# Autodesk Inventor assembly: Asta_verticale
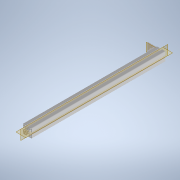
[picture p0: Inventor's stored thumbnail of the model, 180x180]
Saved by Autodesk Inventor 2022 (Build 260153000, 153)
## iProperties
Created: 2022-02-11
Part Number: Asta_verticale
Document SubType Name: Assembly
Designer: matte
Author: matte
## Documents named in this file (3)
- C:\Users\matte\Documents\GitHub\MDM-CyberOrto-CAD\Assiemi\Asta_verticale.iam
- C:\Users\matte\Documents\GitHub\MDM-CyberOrto-CAD\Pezzi singoli\Torretta\10-540.ipt
- C:\Users\matte\Documents\GitHub\MDM-CyberOrto-CAD\Parker components\03-Brackets_Gussets_Plates\08-Angle Brackets\28-602.ipt
## Components (2 placed, 2 different names)
1. 10-540:1 — Coincidente:1, Allineato:1, Coincidente:2
2. 28-602:1 — Coincidente:1, Allineato:1, Coincidente:2, Coincidente:3, Angolo:1
## Relationships (5: Mate 3, Flush 1, Angle 1)
- Coincidente:1 [Mate]: 10-540:1 ↔ 28-602:1
- Allineato:1 [Flush]: 10-540:1 ↔ 28-602:1
- Coincidente:2 [Mate]: 10-540:1 ↔ 28-602:1
- Coincidente:3 [Mate]: 28-602:1
- Angolo:1 [Angle] (0 deg): 28-602:1
